(part 1 of 2)
# Autodesk Inventor assembly: Raspberry Pi 3
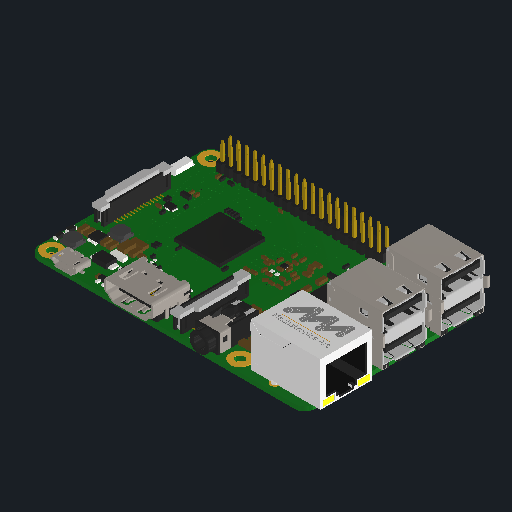
[picture p0: Inventor's stored thumbnail of the model, 512x512]
Saved by Autodesk Inventor 2023 (Build 270158000, 158)
## iProperties
Created: 2016-12-17
Part Number: Raspberry Pi 3
Description: STEP AP214
Document SubType Name: Assembly
Designer: Manuel
Sending System: SolidWorks 2016
Preprocessor: SwSTEP 2.0
Title: Raspberry Pi 3.STEP
Revision Number: ANY
## Documents named in this file (328)
- C:\workspace\Studium\WST\opcua_netzwerk\Entwicklung Knoten\3D Modell\Raspberry Pi 3B\Raspberry Pi 3.iam
- C:\workspace\Studium\WST\opcua_netzwerk\Entwicklung Knoten\3D Modell\Raspberry Pi 3B\Raspberry Pi 3157.ipt
- C:\workspace\Studium\WST\opcua_netzwerk\Entwicklung Knoten\3D Modell\Raspberry Pi 3B\Raspberry Pi 3242.ipt
- C:\workspace\Studium\WST\opcua_netzwerk\Entwicklung Knoten\3D Modell\Raspberry Pi 3B\Raspberry Pi 3266.ipt
- C:\workspace\Studium\WST\opcua_netzwerk\Entwicklung Knoten\3D Modell\Raspberry Pi 3B\raspberry_pi_3(bar_180_2x20).ipt
- C:\workspace\Studium\WST\opcua_netzwerk\Entwicklung Knoten\3D Modell\Raspberry Pi 3B\RPi3_ModelB v1.iam
- C:\workspace\Studium\WST\opcua_netzwerk\Entwicklung Knoten\3D Modell\Raspberry Pi 3B\Raspberry Pi 312.ipt
- C:\workspace\Studium\WST\opcua_netzwerk\Entwicklung Knoten\3D Modell\Raspberry Pi 3B\Raspberry Pi 314.ipt
- C:\workspace\Studium\WST\opcua_netzwerk\Entwicklung Knoten\3D Modell\Raspberry Pi 3B\Raspberry Pi 3172.ipt
- C:\workspace\Studium\WST\opcua_netzwerk\Entwicklung Knoten\3D Modell\Raspberry Pi 3B\Raspberry Pi 3173.ipt
- C:\workspace\Studium\WST\opcua_netzwerk\Entwicklung Knoten\3D Modell\Raspberry Pi 3B\Raspberry Pi 3174.ipt
- C:\workspace\Studium\WST\opcua_netzwerk\Entwicklung Knoten\3D Modell\Raspberry Pi 3B\Raspberry Pi 3175.ipt
- C:\workspace\Studium\WST\opcua_netzwerk\Entwicklung Knoten\3D Modell\Raspberry Pi 3B\Raspberry Pi 3176.ipt
- C:\workspace\Studium\WST\opcua_netzwerk\Entwicklung Knoten\3D Modell\Raspberry Pi 3B\Raspberry Pi 3177.ipt
- C:\workspace\Studium\WST\opcua_netzwerk\Entwicklung Knoten\3D Modell\Raspberry Pi 3B\Raspberry Pi 3178.ipt
- C:\workspace\Studium\WST\opcua_netzwerk\Entwicklung Knoten\3D Modell\Raspberry Pi 3B\Raspberry Pi 3179.ipt
- C:\workspace\Studium\WST\opcua_netzwerk\Entwicklung Knoten\3D Modell\Raspberry Pi 3B\Raspberry Pi 3180.ipt
- C:\workspace\Studium\WST\opcua_netzwerk\Entwicklung Knoten\3D Modell\Raspberry Pi 3B\Raspberry Pi 3181.ipt
- C:\workspace\Studium\WST\opcua_netzwerk\Entwicklung Knoten\3D Modell\Raspberry Pi 3B\Raspberry Pi 3182.ipt
- C:\workspace\Studium\WST\opcua_netzwerk\Entwicklung Knoten\3D Modell\Raspberry Pi 3B\Raspberry Pi 3183.ipt
- C:\workspace\Studium\WST\opcua_netzwerk\Entwicklung Knoten\3D Modell\Raspberry Pi 3B\Raspberry Pi 3184.ipt
- C:\workspace\Studium\WST\opcua_netzwerk\Entwicklung Knoten\3D Modell\Raspberry Pi 3B\Raspberry Pi 3185.ipt
- C:\workspace\Studium\WST\opcua_netzwerk\Entwicklung Knoten\3D Modell\Raspberry Pi 3B\Raspberry Pi 3186.ipt
- C:\workspace\Studium\WST\opcua_netzwerk\Entwicklung Knoten\3D Modell\Raspberry Pi 3B\Raspberry Pi 3187.ipt
- C:\workspace\Studium\WST\opcua_netzwerk\Entwicklung Knoten\3D Modell\Raspberry Pi 3B\Raspberry Pi 3188.ipt
- C:\workspace\Studium\WST\opcua_netzwerk\Entwicklung Knoten\3D Modell\Raspberry Pi 3B\Raspberry Pi 3189.ipt
- C:\workspace\Studium\WST\opcua_netzwerk\Entwicklung Knoten\3D Modell\Raspberry Pi 3B\Raspberry Pi 3190.ipt
- C:\workspace\Studium\WST\opcua_netzwerk\Entwicklung Knoten\3D Modell\Raspberry Pi 3B\Raspberry Pi 3191.ipt
- C:\workspace\Studium\WST\opcua_netzwerk\Entwicklung Knoten\3D Modell\Raspberry Pi 3B\Raspberry Pi 3192.ipt
- C:\workspace\Studium\WST\opcua_netzwerk\Entwicklung Knoten\3D Modell\Raspberry Pi 3B\Raspberry Pi 3193.ipt
- C:\workspace\Studium\WST\opcua_netzwerk\Entwicklung Knoten\3D Modell\Raspberry Pi 3B\Raspberry Pi 3194.ipt
- C:\workspace\Studium\WST\opcua_netzwerk\Entwicklung Knoten\3D Modell\Raspberry Pi 3B\Raspberry Pi 3195.ipt
- C:\workspace\Studium\WST\opcua_netzwerk\Entwicklung Knoten\3D Modell\Raspberry Pi 3B\Raspberry Pi 3196.ipt
- C:\workspace\Studium\WST\opcua_netzwerk\Entwicklung Knoten\3D Modell\Raspberry Pi 3B\Raspberry Pi 3197.ipt
- C:\workspace\Studium\WST\opcua_netzwerk\Entwicklung Knoten\3D Modell\Raspberry Pi 3B\Raspberry Pi 3198.ipt
- C:\workspace\Studium\WST\opcua_netzwerk\Entwicklung Knoten\3D Modell\Raspberry Pi 3B\Raspberry Pi 3199.ipt
- C:\workspace\Studium\WST\opcua_netzwerk\Entwicklung Knoten\3D Modell\Raspberry Pi 3B\Raspberry Pi 3200.ipt
- C:\workspace\Studium\WST\opcua_netzwerk\Entwicklung Knoten\3D Modell\Raspberry Pi 3B\Raspberry Pi 3201.ipt
- C:\workspace\Studium\WST\opcua_netzwerk\Entwicklung Knoten\3D Modell\Raspberry Pi 3B\Raspberry Pi 3202.ipt
- C:\workspace\Studium\WST\opcua_netzwerk\Entwicklung Knoten\3D Modell\Raspberry Pi 3B\Raspberry Pi 3203.ipt
- C:\workspace\Studium\WST\opcua_netzwerk\Entwicklung Knoten\3D Modell\Raspberry Pi 3B\Raspberry Pi 3204.ipt
- C:\workspace\Studium\WST\opcua_netzwerk\Entwicklung Knoten\3D Modell\Raspberry Pi 3B\Raspberry Pi 3205.ipt
- C:\workspace\Studium\WST\opcua_netzwerk\Entwicklung Knoten\3D Modell\Raspberry Pi 3B\Raspberry Pi 3206.ipt
- C:\workspace\Studium\WST\opcua_netzwerk\Entwicklung Knoten\3D Modell\Raspberry Pi 3B\Raspberry Pi 3207.ipt
- C:\workspace\Studium\WST\opcua_netzwerk\Entwicklung Knoten\3D Modell\Raspberry Pi 3B\Raspberry Pi 3208.ipt
- C:\workspace\Studium\WST\opcua_netzwerk\Entwicklung Knoten\3D Modell\Raspberry Pi 3B\Raspberry Pi 3209.ipt
- C:\workspace\Studium\WST\opcua_netzwerk\Entwicklung Knoten\3D Modell\Raspberry Pi 3B\Raspberry Pi 3210.ipt
- C:\workspace\Studium\WST\opcua_netzwerk\Entwicklung Knoten\3D Modell\Raspberry Pi 3B\Raspberry Pi 3211.ipt
- C:\workspace\Studium\WST\opcua_netzwerk\Entwicklung Knoten\3D Modell\Raspberry Pi 3B\Raspberry Pi 3212.ipt
- C:\workspace\Studium\WST\opcua_netzwerk\Entwicklung Knoten\3D Modell\Raspberry Pi 3B\Raspberry Pi 3213.ipt
- C:\workspace\Studium\WST\opcua_netzwerk\Entwicklung Knoten\3D Modell\Raspberry Pi 3B\Raspberry Pi 3214.ipt
- C:\workspace\Studium\WST\opcua_netzwerk\Entwicklung Knoten\3D Modell\Raspberry Pi 3B\Raspberry Pi 3215.ipt
- C:\workspace\Studium\WST\opcua_netzwerk\Entwicklung Knoten\3D Modell\Raspberry Pi 3B\Raspberry Pi 3216.ipt
- C:\workspace\Studium\WST\opcua_netzwerk\Entwicklung Knoten\3D Modell\Raspberry Pi 3B\Raspberry Pi 3217.ipt
- C:\workspace\Studium\WST\opcua_netzwerk\Entwicklung Knoten\3D Modell\Raspberry Pi 3B\Raspberry Pi 3218.ipt
- C:\workspace\Studium\WST\opcua_netzwerk\Entwicklung Knoten\3D Modell\Raspberry Pi 3B\Raspberry Pi 3219.ipt
- C:\workspace\Studium\WST\opcua_netzwerk\Entwicklung Knoten\3D Modell\Raspberry Pi 3B\Raspberry Pi 3220.ipt
- C:\workspace\Studium\WST\opcua_netzwerk\Entwicklung Knoten\3D Modell\Raspberry Pi 3B\Raspberry Pi 3221.ipt
- C:\workspace\Studium\WST\opcua_netzwerk\Entwicklung Knoten\3D Modell\Raspberry Pi 3B\Raspberry Pi 3222.ipt
- C:\workspace\Studium\WST\opcua_netzwerk\Entwicklung Knoten\3D Modell\Raspberry Pi 3B\Raspberry Pi 3223.ipt
- C:\workspace\Studium\WST\opcua_netzwerk\Entwicklung Knoten\3D Modell\Raspberry Pi 3B\Raspberry Pi 3224.ipt
- C:\workspace\Studium\WST\opcua_netzwerk\Entwicklung Knoten\3D Modell\Raspberry Pi 3B\Raspberry Pi 3225.ipt
- C:\workspace\Studium\WST\opcua_netzwerk\Entwicklung Knoten\3D Modell\Raspberry Pi 3B\Raspberry Pi 3226.ipt
- C:\workspace\Studium\WST\opcua_netzwerk\Entwicklung Knoten\3D Modell\Raspberry Pi 3B\Raspberry Pi 3227.ipt
- C:\workspace\Studium\WST\opcua_netzwerk\Entwicklung Knoten\3D Modell\Raspberry Pi 3B\Raspberry Pi 3228.ipt
- C:\workspace\Studium\WST\opcua_netzwerk\Entwicklung Knoten\3D Modell\Raspberry Pi 3B\Raspberry Pi 3229.ipt
- C:\workspace\Studium\WST\opcua_netzwerk\Entwicklung Knoten\3D Modell\Raspberry Pi 3B\Raspberry Pi 3230.ipt
- C:\workspace\Studium\WST\opcua_netzwerk\Entwicklung Knoten\3D Modell\Raspberry Pi 3B\Raspberry Pi 3231.ipt
- C:\workspace\Studium\WST\opcua_netzwerk\Entwicklung Knoten\3D Modell\Raspberry Pi 3B\Raspberry Pi 3232.ipt
- C:\workspace\Studium\WST\opcua_netzwerk\Entwicklung Knoten\3D Modell\Raspberry Pi 3B\Raspberry Pi 3233.ipt
- C:\workspace\Studium\WST\opcua_netzwerk\Entwicklung Knoten\3D Modell\Raspberry Pi 3B\Raspberry Pi 3234.ipt
- C:\workspace\Studium\WST\opcua_netzwerk\Entwicklung Knoten\3D Modell\Raspberry Pi 3B\Raspberry Pi 3235.ipt
- C:\workspace\Studium\WST\opcua_netzwerk\Entwicklung Knoten\3D Modell\Raspberry Pi 3B\Raspberry Pi 31.ipt
- C:\workspace\Studium\WST\opcua_netzwerk\Entwicklung Knoten\3D Modell\Raspberry Pi 3B\Raspberry Pi 32.ipt
- C:\workspace\Studium\WST\opcua_netzwerk\Entwicklung Knoten\3D Modell\Raspberry Pi 3B\Raspberry Pi 33.ipt
- C:\workspace\Studium\WST\opcua_netzwerk\Entwicklung Knoten\3D Modell\Raspberry Pi 3B\Raspberry Pi 34.ipt
- C:\workspace\Studium\WST\opcua_netzwerk\Entwicklung Knoten\3D Modell\Raspberry Pi 3B\Raspberry Pi 35.ipt
- C:\workspace\Studium\WST\opcua_netzwerk\Entwicklung Knoten\3D Modell\Raspberry Pi 3B\Raspberry Pi 36.ipt
- C:\workspace\Studium\WST\opcua_netzwerk\Entwicklung Knoten\3D Modell\Raspberry Pi 3B\Raspberry Pi 37.ipt
- C:\workspace\Studium\WST\opcua_netzwerk\Entwicklung Knoten\3D Modell\Raspberry Pi 3B\Raspberry Pi 38.ipt
- C:\workspace\Studium\WST\opcua_netzwerk\Entwicklung Knoten\3D Modell\Raspberry Pi 3B\Raspberry Pi 39.ipt
- C:\workspace\Studium\WST\opcua_netzwerk\Entwicklung Knoten\3D Modell\Raspberry Pi 3B\Raspberry Pi 310.ipt
- C:\workspace\Studium\WST\opcua_netzwerk\Entwicklung Knoten\3D Modell\Raspberry Pi 3B\Raspberry Pi 311.ipt
- C:\workspace\Studium\WST\opcua_netzwerk\Entwicklung Knoten\3D Modell\Raspberry Pi 3B\Raspberry Pi 313.ipt
- C:\workspace\Studium\WST\opcua_netzwerk\Entwicklung Knoten\3D Modell\Raspberry Pi 3B\Raspberry Pi 315.ipt
- C:\workspace\Studium\WST\opcua_netzwerk\Entwicklung Knoten\3D Modell\Raspberry Pi 3B\Raspberry Pi 316.ipt
- C:\workspace\Studium\WST\opcua_netzwerk\Entwicklung Knoten\3D Modell\Raspberry Pi 3B\Raspberry Pi 317.ipt
- C:\workspace\Studium\WST\opcua_netzwerk\Entwicklung Knoten\3D Modell\Raspberry Pi 3B\Raspberry Pi 318.ipt
- C:\workspace\Studium\WST\opcua_netzwerk\Entwicklung Knoten\3D Modell\Raspberry Pi 3B\Raspberry Pi 319.ipt
- C:\workspace\Studium\WST\opcua_netzwerk\Entwicklung Knoten\3D Modell\Raspberry Pi 3B\Raspberry Pi 320.ipt
- C:\workspace\Studium\WST\opcua_netzwerk\Entwicklung Knoten\3D Modell\Raspberry Pi 3B\Raspberry Pi 322.ipt
- C:\workspace\Studium\WST\opcua_netzwerk\Entwicklung Knoten\3D Modell\Raspberry Pi 3B\Raspberry Pi 323.ipt
- C:\workspace\Studium\WST\opcua_netzwerk\Entwicklung Knoten\3D Modell\Raspberry Pi 3B\Raspberry Pi 324.ipt
- C:\workspace\Studium\WST\opcua_netzwerk\Entwicklung Knoten\3D Modell\Raspberry Pi 3B\Raspberry Pi 325.ipt
- C:\workspace\Studium\WST\opcua_netzwerk\Entwicklung Knoten\3D Modell\Raspberry Pi 3B\Raspberry Pi 326.ipt
- C:\workspace\Studium\WST\opcua_netzwerk\Entwicklung Knoten\3D Modell\Raspberry Pi 3B\Raspberry Pi 327.ipt
- C:\workspace\Studium\WST\opcua_netzwerk\Entwicklung Knoten\3D Modell\Raspberry Pi 3B\Raspberry Pi 328.ipt
- C:\workspace\Studium\WST\opcua_netzwerk\Entwicklung Knoten\3D Modell\Raspberry Pi 3B\Raspberry Pi 329.ipt
- C:\workspace\Studium\WST\opcua_netzwerk\Entwicklung Knoten\3D Modell\Raspberry Pi 3B\Raspberry Pi 330.ipt
- C:\workspace\Studium\WST\opcua_netzwerk\Entwicklung Knoten\3D Modell\Raspberry Pi 3B\Raspberry Pi 331.ipt
- C:\workspace\Studium\WST\opcua_netzwerk\Entwicklung Knoten\3D Modell\Raspberry Pi 3B\Raspberry Pi 332.ipt
- C:\workspace\Studium\WST\opcua_netzwerk\Entwicklung Knoten\3D Modell\Raspberry Pi 3B\Raspberry Pi 333.ipt
- C:\workspace\Studium\WST\opcua_netzwerk\Entwicklung Knoten\3D Modell\Raspberry Pi 3B\Raspberry Pi 334.ipt
- C:\workspace\Studium\WST\opcua_netzwerk\Entwicklung Knoten\3D Modell\Raspberry Pi 3B\Raspberry Pi 335.ipt
- C:\workspace\Studium\WST\opcua_netzwerk\Entwicklung Knoten\3D Modell\Raspberry Pi 3B\Raspberry Pi 336.ipt
- C:\workspace\Studium\WST\opcua_netzwerk\Entwicklung Knoten\3D Modell\Raspberry Pi 3B\Raspberry Pi 337.ipt
- C:\workspace\Studium\WST\opcua_netzwerk\Entwicklung Knoten\3D Modell\Raspberry Pi 3B\Raspberry Pi 338.ipt
- C:\workspace\Studium\WST\opcua_netzwerk\Entwicklung Knoten\3D Modell\Raspberry Pi 3B\Raspberry Pi 339.ipt
- C:\workspace\Studium\WST\opcua_netzwerk\Entwicklung Knoten\3D Modell\Raspberry Pi 3B\Raspberry Pi 340.ipt
- C:\workspace\Studium\WST\opcua_netzwerk\Entwicklung Knoten\3D Modell\Raspberry Pi 3B\Raspberry Pi 341.ipt
- C:\workspace\Studium\WST\opcua_netzwerk\Entwicklung Knoten\3D Modell\Raspberry Pi 3B\Raspberry Pi 342.ipt
- C:\workspace\Studium\WST\opcua_netzwerk\Entwicklung Knoten\3D Modell\Raspberry Pi 3B\Raspberry Pi 343.ipt
- C:\workspace\Studium\WST\opcua_netzwerk\Entwicklung Knoten\3D Modell\Raspberry Pi 3B\Raspberry Pi 344.ipt
- C:\workspace\Studium\WST\opcua_netzwerk\Entwicklung Knoten\3D Modell\Raspberry Pi 3B\Raspberry Pi 345.ipt
- C:\workspace\Studium\WST\opcua_netzwerk\Entwicklung Knoten\3D Modell\Raspberry Pi 3B\Raspberry Pi 346.ipt
- C:\workspace\Studium\WST\opcua_netzwerk\Entwicklung Knoten\3D Modell\Raspberry Pi 3B\Raspberry Pi 347.ipt
- C:\workspace\Studium\WST\opcua_netzwerk\Entwicklung Knoten\3D Modell\Raspberry Pi 3B\Raspberry Pi 348.ipt
- C:\workspace\Studium\WST\opcua_netzwerk\Entwicklung Knoten\3D Modell\Raspberry Pi 3B\Raspberry Pi 349.ipt
- C:\workspace\Studium\WST\opcua_netzwerk\Entwicklung Knoten\3D Modell\Raspberry Pi 3B\Raspberry Pi 350.ipt
- C:\workspace\Studium\WST\opcua_netzwerk\Entwicklung Knoten\3D Modell\Raspberry Pi 3B\Raspberry Pi 351.ipt
- C:\workspace\Studium\WST\opcua_netzwerk\Entwicklung Knoten\3D Modell\Raspberry Pi 3B\Raspberry Pi 352.ipt
- C:\workspace\Studium\WST\opcua_netzwerk\Entwicklung Knoten\3D Modell\Raspberry Pi 3B\Raspberry Pi 353.ipt
- C:\workspace\Studium\WST\opcua_netzwerk\Entwicklung Knoten\3D Modell\Raspberry Pi 3B\Raspberry Pi 354.ipt
- C:\workspace\Studium\WST\opcua_netzwerk\Entwicklung Knoten\3D Modell\Raspberry Pi 3B\Raspberry Pi 355.ipt
- C:\workspace\Studium\WST\opcua_netzwerk\Entwicklung Knoten\3D Modell\Raspberry Pi 3B\Raspberry Pi 356.ipt
- C:\workspace\Studium\WST\opcua_netzwerk\Entwicklung Knoten\3D Modell\Raspberry Pi 3B\Raspberry Pi 357.ipt
- C:\workspace\Studium\WST\opcua_netzwerk\Entwicklung Knoten\3D Modell\Raspberry Pi 3B\Raspberry Pi 358.ipt
- C:\workspace\Studium\WST\opcua_netzwerk\Entwicklung Knoten\3D Modell\Raspberry Pi 3B\Raspberry Pi 359.ipt
- C:\workspace\Studium\WST\opcua_netzwerk\Entwicklung Knoten\3D Modell\Raspberry Pi 3B\Raspberry Pi 360.ipt
- C:\workspace\Studium\WST\opcua_netzwerk\Entwicklung Knoten\3D Modell\Raspberry Pi 3B\Raspberry Pi 361.ipt
- C:\workspace\Studium\WST\opcua_netzwerk\Entwicklung Knoten\3D Modell\Raspberry Pi 3B\Raspberry Pi 362.ipt
- C:\workspace\Studium\WST\opcua_netzwerk\Entwicklung Knoten\3D Modell\Raspberry Pi 3B\Raspberry Pi 363.ipt
- C:\workspace\Studium\WST\opcua_netzwerk\Entwicklung Knoten\3D Modell\Raspberry Pi 3B\Raspberry Pi 364.ipt
- C:\workspace\Studium\WST\opcua_netzwerk\Entwicklung Knoten\3D Modell\Raspberry Pi 3B\Raspberry Pi 365.ipt
- C:\workspace\Studium\WST\opcua_netzwerk\Entwicklung Knoten\3D Modell\Raspberry Pi 3B\Raspberry Pi 366.ipt
- C:\workspace\Studium\WST\opcua_netzwerk\Entwicklung Knoten\3D Modell\Raspberry Pi 3B\Raspberry Pi 367.ipt
- C:\workspace\Studium\WST\opcua_netzwerk\Entwicklung Knoten\3D Modell\Raspberry Pi 3B\Raspberry Pi 368.ipt
- C:\workspace\Studium\WST\opcua_netzwerk\Entwicklung Knoten\3D Modell\Raspberry Pi 3B\Raspberry Pi 369.ipt
- C:\workspace\Studium\WST\opcua_netzwerk\Entwicklung Knoten\3D Modell\Raspberry Pi 3B\Raspberry Pi 370.ipt
- C:\workspace\Studium\WST\opcua_netzwerk\Entwicklung Knoten\3D Modell\Raspberry Pi 3B\Raspberry Pi 371.ipt
- C:\workspace\Studium\WST\opcua_netzwerk\Entwicklung Knoten\3D Modell\Raspberry Pi 3B\Raspberry Pi 372.ipt
- C:\workspace\Studium\WST\opcua_netzwerk\Entwicklung Knoten\3D Modell\Raspberry Pi 3B\Raspberry Pi 373.ipt
- C:\workspace\Studium\WST\opcua_netzwerk\Entwicklung Knoten\3D Modell\Raspberry Pi 3B\Raspberry Pi 374.ipt
- C:\workspace\Studium\WST\opcua_netzwerk\Entwicklung Knoten\3D Modell\Raspberry Pi 3B\Raspberry Pi 375.ipt
- C:\workspace\Studium\WST\opcua_netzwerk\Entwicklung Knoten\3D Modell\Raspberry Pi 3B\Raspberry Pi 376.ipt
- C:\workspace\Studium\WST\opcua_netzwerk\Entwicklung Knoten\3D Modell\Raspberry Pi 3B\Raspberry Pi 377.ipt
- C:\workspace\Studium\WST\opcua_netzwerk\Entwicklung Knoten\3D Modell\Raspberry Pi 3B\Raspberry Pi 378.ipt
- C:\workspace\Studium\WST\opcua_netzwerk\Entwicklung Knoten\3D Modell\Raspberry Pi 3B\Raspberry Pi 379.ipt
- C:\workspace\Studium\WST\opcua_netzwerk\Entwicklung Knoten\3D Modell\Raspberry Pi 3B\Raspberry Pi 380.ipt
- C:\workspace\Studium\WST\opcua_netzwerk\Entwicklung Knoten\3D Modell\Raspberry Pi 3B\Raspberry Pi 381.ipt
- C:\workspace\Studium\WST\opcua_netzwerk\Entwicklung Knoten\3D Modell\Raspberry Pi 3B\Raspberry Pi 382.ipt
- C:\workspace\Studium\WST\opcua_netzwerk\Entwicklung Knoten\3D Modell\Raspberry Pi 3B\Raspberry Pi 383.ipt
- C:\workspace\Studium\WST\opcua_netzwerk\Entwicklung Knoten\3D Modell\Raspberry Pi 3B\Raspberry Pi 385.ipt
- C:\workspace\Studium\WST\opcua_netzwerk\Entwicklung Knoten\3D Modell\Raspberry Pi 3B\Raspberry Pi 386.ipt
- C:\workspace\Studium\WST\opcua_netzwerk\Entwicklung Knoten\3D Modell\Raspberry Pi 3B\Raspberry Pi 387.ipt
- C:\workspace\Studium\WST\opcua_netzwerk\Entwicklung Knoten\3D Modell\Raspberry Pi 3B\Raspberry Pi 388.ipt
- C:\workspace\Studium\WST\opcua_netzwerk\Entwicklung Knoten\3D Modell\Raspberry Pi 3B\Raspberry Pi 390.ipt
- C:\workspace\Studium\WST\opcua_netzwerk\Entwicklung Knoten\3D Modell\Raspberry Pi 3B\Raspberry Pi 391.ipt
- C:\workspace\Studium\WST\opcua_netzwerk\Entwicklung Knoten\3D Modell\Raspberry Pi 3B\Raspberry Pi 393.ipt
- C:\workspace\Studium\WST\opcua_netzwerk\Entwicklung Knoten\3D Modell\Raspberry Pi 3B\Raspberry Pi 394.ipt
- C:\workspace\Studium\WST\opcua_netzwerk\Entwicklung Knoten\3D Modell\Raspberry Pi 3B\Raspberry Pi 395.ipt
- C:\workspace\Studium\WST\opcua_netzwerk\Entwicklung Knoten\3D Modell\Raspberry Pi 3B\Raspberry Pi 396.ipt
- C:\workspace\Studium\WST\opcua_netzwerk\Entwicklung Knoten\3D Modell\Raspberry Pi 3B\Raspberry Pi 397.ipt
- C:\workspace\Studium\WST\opcua_netzwerk\Entwicklung Knoten\3D Modell\Raspberry Pi 3B\Raspberry Pi 398.ipt
- C:\workspace\Studium\WST\opcua_netzwerk\Entwicklung Knoten\3D Modell\Raspberry Pi 3B\Raspberry Pi 399.ipt
- C:\workspace\Studium\WST\opcua_netzwerk\Entwicklung Knoten\3D Modell\Raspberry Pi 3B\Raspberry Pi 3100.ipt
- C:\workspace\Studium\WST\opcua_netzwerk\Entwicklung Knoten\3D Modell\Raspberry Pi 3B\Raspberry Pi 3101.ipt
- C:\workspace\Studium\WST\opcua_netzwerk\Entwicklung Knoten\3D Modell\Raspberry Pi 3B\Raspberry Pi 3102.ipt
- C:\workspace\Studium\WST\opcua_netzwerk\Entwicklung Knoten\3D Modell\Raspberry Pi 3B\Raspberry Pi 3103.ipt
- C:\workspace\Studium\WST\opcua_netzwerk\Entwicklung Knoten\3D Modell\Raspberry Pi 3B\Raspberry Pi 3104.ipt
- C:\workspace\Studium\WST\opcua_netzwerk\Entwicklung Knoten\3D Modell\Raspberry Pi 3B\Raspberry Pi 3105.ipt
- C:\workspace\Studium\WST\opcua_netzwerk\Entwicklung Knoten\3D Modell\Raspberry Pi 3B\Raspberry Pi 3106.ipt
- C:\workspace\Studium\WST\opcua_netzwerk\Entwicklung Knoten\3D Modell\Raspberry Pi 3B\Raspberry Pi 3107.ipt
- C:\workspace\Studium\WST\opcua_netzwerk\Entwicklung Knoten\3D Modell\Raspberry Pi 3B\Raspberry Pi 3108.ipt
- C:\workspace\Studium\WST\opcua_netzwerk\Entwicklung Knoten\3D Modell\Raspberry Pi 3B\Raspberry Pi 3109.ipt
- C:\workspace\Studium\WST\opcua_netzwerk\Entwicklung Knoten\3D Modell\Raspberry Pi 3B\Raspberry Pi 3110.ipt
- C:\workspace\Studium\WST\opcua_netzwerk\Entwicklung Knoten\3D Modell\Raspberry Pi 3B\Raspberry Pi 3111.ipt
- C:\workspace\Studium\WST\opcua_netzwerk\Entwicklung Knoten\3D Modell\Raspberry Pi 3B\Raspberry Pi 3112.ipt
- C:\workspace\Studium\WST\opcua_netzwerk\Entwicklung Knoten\3D Modell\Raspberry Pi 3B\Raspberry Pi 3113.ipt
- C:\workspace\Studium\WST\opcua_netzwerk\Entwicklung Knoten\3D Modell\Raspberry Pi 3B\Raspberry Pi 3114.ipt
- C:\workspace\Studium\WST\opcua_netzwerk\Entwicklung Knoten\3D Modell\Raspberry Pi 3B\Raspberry Pi 3115.ipt
- C:\workspace\Studium\WST\opcua_netzwerk\Entwicklung Knoten\3D Modell\Raspberry Pi 3B\Raspberry Pi 3116.ipt
- C:\workspace\Studium\WST\opcua_netzwerk\Entwicklung Knoten\3D Modell\Raspberry Pi 3B\Raspberry Pi 3117.ipt
- C:\workspace\Studium\WST\opcua_netzwerk\Entwicklung Knoten\3D Modell\Raspberry Pi 3B\Raspberry Pi 3118.ipt
- C:\workspace\Studium\WST\opcua_netzwerk\Entwicklung Knoten\3D Modell\Raspberry Pi 3B\Raspberry Pi 3119.ipt
- C:\workspace\Studium\WST\opcua_netzwerk\Entwicklung Knoten\3D Modell\Raspberry Pi 3B\Raspberry Pi 3120.ipt
- C:\workspace\Studium\WST\opcua_netzwerk\Entwicklung Knoten\3D Modell\Raspberry Pi 3B\Raspberry Pi 3121.ipt
- C:\workspace\Studium\WST\opcua_netzwerk\Entwicklung Knoten\3D Modell\Raspberry Pi 3B\Raspberry Pi 3122.ipt
- C:\workspace\Studium\WST\opcua_netzwerk\Entwicklung Knoten\3D Modell\Raspberry Pi 3B\Raspberry Pi 3123.ipt
- C:\workspace\Studium\WST\opcua_netzwerk\Entwicklung Knoten\3D Modell\Raspberry Pi 3B\Raspberry Pi 3124.ipt
- C:\workspace\Studium\WST\opcua_netzwerk\Entwicklung Knoten\3D Modell\Raspberry Pi 3B\Raspberry Pi 3125.ipt
- C:\workspace\Studium\WST\opcua_netzwerk\Entwicklung Knoten\3D Modell\Raspberry Pi 3B\Raspberry Pi 3126.ipt
- C:\workspace\Studium\WST\opcua_netzwerk\Entwicklung Knoten\3D Modell\Raspberry Pi 3B\Raspberry Pi 3127.ipt
- C:\workspace\Studium\WST\opcua_netzwerk\Entwicklung Knoten\3D Modell\Raspberry Pi 3B\Raspberry Pi 3128.ipt
- C:\workspace\Studium\WST\opcua_netzwerk\Entwicklung Knoten\3D Modell\Raspberry Pi 3B\Raspberry Pi 3129.ipt
- C:\workspace\Studium\WST\opcua_netzwerk\Entwicklung Knoten\3D Modell\Raspberry Pi 3B\Raspberry Pi 3130.ipt
- C:\workspace\Studium\WST\opcua_netzwerk\Entwicklung Knoten\3D Modell\Raspberry Pi 3B\Raspberry Pi 3131.ipt
- C:\workspace\Studium\WST\opcua_netzwerk\Entwicklung Knoten\3D Modell\Raspberry Pi 3B\Raspberry Pi 3132.ipt
- C:\workspace\Studium\WST\opcua_netzwerk\Entwicklung Knoten\3D Modell\Raspberry Pi 3B\Raspberry Pi 3133.ipt
- C:\workspace\Studium\WST\opcua_netzwerk\Entwicklung Knoten\3D Modell\Raspberry Pi 3B\Raspberry Pi 3134.ipt
- C:\workspace\Studium\WST\opcua_netzwerk\Entwicklung Knoten\3D Modell\Raspberry Pi 3B\Raspberry Pi 3135.ipt
- C:\workspace\Studium\WST\opcua_netzwerk\Entwicklung Knoten\3D Modell\Raspberry Pi 3B\Raspberry Pi 3137.ipt
- C:\workspace\Studium\WST\opcua_netzwerk\Entwicklung Knoten\3D Modell\Raspberry Pi 3B\Raspberry Pi 3138.ipt
- C:\workspace\Studium\WST\opcua_netzwerk\Entwicklung Knoten\3D Modell\Raspberry Pi 3B\Raspberry Pi 3139.ipt
- C:\workspace\Studium\WST\opcua_netzwerk\Entwicklung Knoten\3D Modell\Raspberry Pi 3B\Raspberry Pi 3140.ipt
- C:\workspace\Studium\WST\opcua_netzwerk\Entwicklung Knoten\3D Modell\Raspberry Pi 3B\Raspberry Pi 3141.ipt
- C:\workspace\Studium\WST\opcua_netzwerk\Entwicklung Knoten\3D Modell\Raspberry Pi 3B\Raspberry Pi 3142.ipt
- C:\workspace\Studium\WST\opcua_netzwerk\Entwicklung Knoten\3D Modell\Raspberry Pi 3B\Raspberry Pi 3143.ipt
- C:\workspace\Studium\WST\opcua_netzwerk\Entwicklung Knoten\3D Modell\Raspberry Pi 3B\Raspberry Pi 3144.ipt
- C:\workspace\Studium\WST\opcua_netzwerk\Entwicklung Knoten\3D Modell\Raspberry Pi 3B\Raspberry Pi 3146.ipt
- C:\workspace\Studium\WST\opcua_netzwerk\Entwicklung Knoten\3D Modell\Raspberry Pi 3B\Raspberry Pi 3147.ipt
- C:\workspace\Studium\WST\opcua_netzwerk\Entwicklung Knoten\3D Modell\Raspberry Pi 3B\Raspberry Pi 3149.ipt
- C:\workspace\Studium\WST\opcua_netzwerk\Entwicklung Knoten\3D Modell\Raspberry Pi 3B\Raspberry Pi 3150.ipt
- C:\workspace\Studium\WST\opcua_netzwerk\Entwicklung Knoten\3D Modell\Raspberry Pi 3B\Raspberry Pi 3151.ipt
- C:\workspace\Studium\WST\opcua_netzwerk\Entwicklung Knoten\3D Modell\Raspberry Pi 3B\Raspberry Pi 3152.ipt
- C:\workspace\Studium\WST\opcua_netzwerk\Entwicklung Knoten\3D Modell\Raspberry Pi 3B\Raspberry Pi 3153.ipt
- C:\workspace\Studium\WST\opcua_netzwerk\Entwicklung Knoten\3D Modell\Raspberry Pi 3B\Raspberry Pi 3154.ipt
- C:\workspace\Studium\WST\opcua_netzwerk\Entwicklung Knoten\3D Modell\Raspberry Pi 3B\Raspberry Pi 3155.ipt
- C:\workspace\Studium\WST\opcua_netzwerk\Entwicklung Knoten\3D Modell\Raspberry Pi 3B\Raspberry Pi 3156.ipt
- C:\workspace\Studium\WST\opcua_netzwerk\Entwicklung Knoten\3D Modell\Raspberry Pi 3B\Raspberry Pi 3158.ipt
- C:\workspace\Studium\WST\opcua_netzwerk\Entwicklung Knoten\3D Modell\Raspberry Pi 3B\Raspberry Pi 3159.ipt
- C:\workspace\Studium\WST\opcua_netzwerk\Entwicklung Knoten\3D Modell\Raspberry Pi 3B\Raspberry Pi 3160.ipt
- C:\workspace\Studium\WST\opcua_netzwerk\Entwicklung Knoten\3D Modell\Raspberry Pi 3B\Raspberry Pi 3161.ipt
- C:\workspace\Studium\WST\opcua_netzwerk\Entwicklung Knoten\3D Modell\Raspberry Pi 3B\Raspberry Pi 3162.ipt
- C:\workspace\Studium\WST\opcua_netzwerk\Entwicklung Knoten\3D Modell\Raspberry Pi 3B\Raspberry Pi 3163.ipt
- C:\workspace\Studium\WST\opcua_netzwerk\Entwicklung Knoten\3D Modell\Raspberry Pi 3B\Raspberry Pi 3164.ipt
- C:\workspace\Studium\WST\opcua_netzwerk\Entwicklung Knoten\3D Modell\Raspberry Pi 3B\Raspberry Pi 3165.ipt
- C:\workspace\Studium\WST\opcua_netzwerk\Entwicklung Knoten\3D Modell\Raspberry Pi 3B\Raspberry Pi 3166.ipt
- C:\workspace\Studium\WST\opcua_netzwerk\Entwicklung Knoten\3D Modell\Raspberry Pi 3B\Raspberry Pi 3167.ipt
- C:\workspace\Studium\WST\opcua_netzwerk\Entwicklung Knoten\3D Modell\Raspberry Pi 3B\Raspberry Pi 3168.ipt
- C:\workspace\Studium\WST\opcua_netzwerk\Entwicklung Knoten\3D Modell\Raspberry Pi 3B\Raspberry Pi 3169.ipt
- C:\workspace\Studium\WST\opcua_netzwerk\Entwicklung Knoten\3D Modell\Raspberry Pi 3B\Raspberry Pi 3170.ipt
- C:\workspace\Studium\WST\opcua_netzwerk\Entwicklung Knoten\3D Modell\Raspberry Pi 3B\Raspberry Pi 3171.ipt
- C:\workspace\Studium\WST\opcua_netzwerk\Entwicklung Knoten\3D Modell\Raspberry Pi 3B\Raspberry Pi 3276.ipt
- C:\workspace\Studium\WST\opcua_netzwerk\Entwicklung Knoten\3D Modell\Raspberry Pi 3B\Raspberry Pi 3277.ipt
- C:\workspace\Studium\WST\opcua_netzwerk\Entwicklung Knoten\3D Modell\Raspberry Pi 3B\Raspberry Pi 3278.ipt
- C:\workspace\Studium\WST\opcua_netzwerk\Entwicklung Knoten\3D Modell\Raspberry Pi 3B\Raspberry Pi 3279.ipt
- C:\workspace\Studium\WST\opcua_netzwerk\Entwicklung Knoten\3D Modell\Raspberry Pi 3B\Raspberry Pi 3280.ipt
- C:\workspace\Studium\WST\opcua_netzwerk\Entwicklung Knoten\3D Modell\Raspberry Pi 3B\Raspberry Pi 3281.ipt
- C:\workspace\Studium\WST\opcua_netzwerk\Entwicklung Knoten\3D Modell\Raspberry Pi 3B\Raspberry Pi 3282.ipt
- C:\workspace\Studium\WST\opcua_netzwerk\Entwicklung Knoten\3D Modell\Raspberry Pi 3B\Raspberry Pi 3283.ipt
- C:\workspace\Studium\WST\opcua_netzwerk\Entwicklung Knoten\3D Modell\Raspberry Pi 3B\Raspberry Pi 3284.ipt
- C:\workspace\Studium\WST\opcua_netzwerk\Entwicklung Knoten\3D Modell\Raspberry Pi 3B\Raspberry Pi 3285.ipt
- C:\workspace\Studium\WST\opcua_netzwerk\Entwicklung Knoten\3D Modell\Raspberry Pi 3B\Raspberry Pi 3286.ipt
- C:\workspace\Studium\WST\opcua_netzwerk\Entwicklung Knoten\3D Modell\Raspberry Pi 3B\Raspberry Pi 3287.ipt
- C:\workspace\Studium\WST\opcua_netzwerk\Entwicklung Knoten\3D Modell\Raspberry Pi 3B\Raspberry Pi 3288.ipt
- C:\workspace\Studium\WST\opcua_netzwerk\Entwicklung Knoten\3D Modell\Raspberry Pi 3B\Raspberry Pi 3289.ipt
- C:\workspace\Studium\WST\opcua_netzwerk\Entwicklung Knoten\3D Modell\Raspberry Pi 3B\Raspberry Pi 3290.ipt
- C:\workspace\Studium\WST\opcua_netzwerk\Entwicklung Knoten\3D Modell\Raspberry Pi 3B\Raspberry Pi 3291.ipt
- C:\workspace\Studium\WST\opcua_netzwerk\Entwicklung Knoten\3D Modell\Raspberry Pi 3B\Raspberry Pi 3292.ipt
- C:\workspace\Studium\WST\opcua_netzwerk\Entwicklung Knoten\3D Modell\Raspberry Pi 3B\Raspberry Pi 3293.ipt
- C:\workspace\Studium\WST\opcua_netzwerk\Entwicklung Knoten\3D Modell\Raspberry Pi 3B\Raspberry Pi 3294.ipt
- C:\workspace\Studium\WST\opcua_netzwerk\Entwicklung Knoten\3D Modell\Raspberry Pi 3B\Raspberry Pi 3295.ipt
- C:\workspace\Studium\WST\opcua_netzwerk\Entwicklung Knoten\3D Modell\Raspberry Pi 3B\Raspberry Pi 3296.ipt
- C:\workspace\Studium\WST\opcua_netzwerk\Entwicklung Knoten\3D Modell\Raspberry Pi 3B\Raspberry Pi 3297.ipt
- C:\workspace\Studium\WST\opcua_netzwerk\Entwicklung Knoten\3D Modell\Raspberry Pi 3B\Raspberry Pi 3298.ipt
- C:\workspace\Studium\WST\opcua_netzwerk\Entwicklung Knoten\3D Modell\Raspberry Pi 3B\Raspberry Pi 3299.ipt
- C:\workspace\Studium\WST\opcua_netzwerk\Entwicklung Knoten\3D Modell\Raspberry Pi 3B\Raspberry Pi 3300.ipt
- C:\workspace\Studium\WST\opcua_netzwerk\Entwicklung Knoten\3D Modell\Raspberry Pi 3B\Raspberry Pi 3301.ipt
- C:\workspace\Studium\WST\opcua_netzwerk\Entwicklung Knoten\3D Modell\Raspberry Pi 3B\Raspberry Pi 3302.ipt
- C:\workspace\Studium\WST\opcua_netzwerk\Entwicklung Knoten\3D Modell\Raspberry Pi 3B\Raspberry Pi 3303.ipt
- C:\workspace\Studium\WST\opcua_netzwerk\Entwicklung Knoten\3D Modell\Raspberry Pi 3B\Raspberry Pi 3304.ipt
- C:\workspace\Studium\WST\opcua_netzwerk\Entwicklung Knoten\3D Modell\Raspberry Pi 3B\Raspberry Pi 3305.ipt
- C:\workspace\Studium\WST\opcua_netzwerk\Entwicklung Knoten\3D Modell\Raspberry Pi 3B\Raspberry Pi 3306.ipt
- C:\workspace\Studium\WST\opcua_netzwerk\Entwicklung Knoten\3D Modell\Raspberry Pi 3B\Raspberry Pi 3307.ipt
- C:\workspace\Studium\WST\opcua_netzwerk\Entwicklung Knoten\3D Modell\Raspberry Pi 3B\Raspberry Pi 3308.ipt
- C:\workspace\Studium\WST\opcua_netzwerk\Entwicklung Knoten\3D Modell\Raspberry Pi 3B\Raspberry Pi 3309.ipt
- C:\workspace\Studium\WST\opcua_netzwerk\Entwicklung Knoten\3D Modell\Raspberry Pi 3B\Raspberry Pi 3310.ipt
- C:\workspace\Studium\WST\opcua_netzwerk\Entwicklung Knoten\3D Modell\Raspberry Pi 3B\Raspberry Pi 3311.ipt
- C:\workspace\Studium\WST\opcua_netzwerk\Entwicklung Knoten\3D Modell\Raspberry Pi 3B\Raspberry Pi 3312.ipt
- C:\workspace\Studium\WST\opcua_netzwerk\Entwicklung Knoten\3D Modell\Raspberry Pi 3B\Raspberry Pi 3313.ipt
- C:\workspace\Studium\WST\opcua_netzwerk\Entwicklung Knoten\3D Modell\Raspberry Pi 3B\Raspberry Pi 3314.ipt
- C:\workspace\Studium\WST\opcua_netzwerk\Entwicklung Knoten\3D Modell\Raspberry Pi 3B\Raspberry Pi 3315.ipt
- C:\workspace\Studium\WST\opcua_netzwerk\Entwicklung Knoten\3D Modell\Raspberry Pi 3B\Raspberry Pi 3316.ipt
- C:\workspace\Studium\WST\opcua_netzwerk\Entwicklung Knoten\3D Modell\Raspberry Pi 3B\Raspberry Pi 3317.ipt
- C:\workspace\Studium\WST\opcua_netzwerk\Entwicklung Knoten\3D Modell\Raspberry Pi 3B\Raspberry Pi 3318.ipt
- C:\workspace\Studium\WST\opcua_netzwerk\Entwicklung Knoten\3D Modell\Raspberry Pi 3B\Raspberry Pi 3319.ipt
- C:\workspace\Studium\WST\opcua_netzwerk\Entwicklung Knoten\3D Modell\Raspberry Pi 3B\Raspberry Pi 3320.ipt
- C:\workspace\Studium\WST\opcua_netzwerk\Entwicklung Knoten\3D Modell\Raspberry Pi 3B\Raspberry Pi 3321.ipt
- C:\workspace\Studium\WST\opcua_netzwerk\Entwicklung Knoten\3D Modell\Raspberry Pi 3B\Raspberry Pi 3322.ipt
- C:\workspace\Studium\WST\opcua_netzwerk\Entwicklung Knoten\3D Modell\Raspberry Pi 3B\Raspberry Pi 3323.ipt
- C:\workspace\Studium\WST\opcua_netzwerk\Entwicklung Knoten\3D Modell\Raspberry Pi 3B\Raspberry Pi 3324.ipt
- C:\workspace\Studium\WST\opcua_netzwerk\Entwicklung Knoten\3D Modell\Raspberry Pi 3B\Raspberry Pi 3325.ipt
- C:\workspace\Studium\WST\opcua_netzwerk\Entwicklung Knoten\3D Modell\Raspberry Pi 3B\Raspberry Pi 3326.ipt
- C:\workspace\Studium\WST\opcua_netzwerk\Entwicklung Knoten\3D Modell\Raspberry Pi 3B\Raspberry Pi 3327.ipt
- C:\workspace\Studium\WST\opcua_netzwerk\Entwicklung Knoten\3D Modell\Raspberry Pi 3B\Raspberry Pi 3328.ipt
- C:\workspace\Studium\WST\opcua_netzwerk\Entwicklung Knoten\3D Modell\Raspberry Pi 3B\Raspberry Pi 3329.ipt
- C:\workspace\Studium\WST\opcua_netzwerk\Entwicklung Knoten\3D Modell\Raspberry Pi 3B\Raspberry Pi 3330.ipt
- C:\workspace\Studium\WST\opcua_netzwerk\Entwicklung Knoten\3D Modell\Raspberry Pi 3B\Raspberry Pi 3331.ipt
- C:\workspace\Studium\WST\opcua_netzwerk\Entwicklung Knoten\3D Modell\Raspberry Pi 3B\Raspberry Pi 3332.ipt
- C:\workspace\Studium\WST\opcua_netzwerk\Entwicklung Knoten\3D Modell\Raspberry Pi 3B\Raspberry Pi 3333.ipt
- C:\workspace\Studium\WST\opcua_netzwerk\Entwicklung Knoten\3D Modell\Raspberry Pi 3B\Raspberry Pi 3334.ipt
- C:\workspace\Studium\WST\opcua_netzwerk\Entwicklung Knoten\3D Modell\Raspberry Pi 3B\Raspberry Pi 3335.ipt
- C:\workspace\Studium\WST\opcua_netzwerk\Entwicklung Knoten\3D Modell\Raspberry Pi 3B\Raspberry Pi 3336.ipt
- C:\workspace\Studium\WST\opcua_netzwerk\Entwicklung Knoten\3D Modell\Raspberry Pi 3B\Raspberry Pi 3337.ipt
- C:\workspace\Studium\WST\opcua_netzwerk\Entwicklung Knoten\3D Modell\Raspberry Pi 3B\Raspberry Pi 3338.ipt
- C:\workspace\Studium\WST\opcua_netzwerk\Entwicklung Knoten\3D Modell\Raspberry Pi 3B\Raspberry Pi 3339.ipt
- C:\workspace\Studium\WST\opcua_netzwerk\Entwicklung Knoten\3D Modell\Raspberry Pi 3B\Raspberry Pi 3340.ipt
- C:\workspace\Studium\WST\opcua_netzwerk\Entwicklung Knoten\3D Modell\Raspberry Pi 3B\Raspberry Pi 3341.ipt
- C:\workspace\Studium\WST\opcua_netzwerk\Entwicklung Knoten\3D Modell\Raspberry Pi 3B\Raspberry Pi 3342.ipt
- C:\workspace\Studium\WST\opcua_netzwerk\Entwicklung Knoten\3D Modell\Raspberry Pi 3B\Raspberry Pi 3343.ipt
- C:\workspace\Studium\WST\opcua_netzwerk\Entwicklung Knoten\3D Modell\Raspberry Pi 3B\Raspberry Pi 3344.ipt
- C:\workspace\Studium\WST\opcua_netzwerk\Entwicklung Knoten\3D Modell\Raspberry Pi 3B\Raspberry Pi 3345.ipt
- C:\workspace\Studium\WST\opcua_netzwerk\Entwicklung Knoten\3D Modell\Raspberry Pi 3B\Raspberry Pi 3346.ipt
- C:\workspace\Studium\WST\opcua_netzwerk\Entwicklung Knoten\3D Modell\Raspberry Pi 3B\Raspberry Pi 3347.ipt
- C:\workspace\Studium\WST\opcua_netzwerk\Entwicklung Knoten\3D Modell\Raspberry Pi 3B\Raspberry Pi 3348.ipt
- C:\workspace\Studium\WST\opcua_netzwerk\Entwicklung Knoten\3D Modell\Raspberry Pi 3B\Raspberry Pi 3349.ipt
- C:\workspace\Studium\WST\opcua_netzwerk\Entwicklung Knoten\3D Modell\Raspberry Pi 3B\Raspberry Pi 3350.ipt
- C:\workspace\Studium\WST\opcua_netzwerk\Entwicklung Knoten\3D Modell\Raspberry Pi 3B\Raspberry Pi 3351.ipt
- C:\workspace\Studium\WST\opcua_netzwerk\Entwicklung Knoten\3D Modell\Raspberry Pi 3B\Raspberry Pi 3352.ipt
- C:\workspace\Studium\WST\opcua_netzwerk\Entwicklung Knoten\3D Modell\Raspberry Pi 3B\Raspberry Pi 3353.ipt
- C:\workspace\Studium\WST\opcua_netzwerk\Entwicklung Knoten\3D Modell\Raspberry Pi 3B\Raspberry Pi 3354.ipt
- C:\workspace\Studium\WST\opcua_netzwerk\Entwicklung Knoten\3D Modell\Raspberry Pi 3B\Raspberry Pi 3357.ipt
- C:\workspace\Studium\WST\opcua_netzwerk\Entwicklung Knoten\3D Modell\Raspberry Pi 3B\Raspberry Pi 3355.ipt
- C:\workspace\Studium\WST\opcua_netzwerk\Entwicklung Knoten\3D Modell\Raspberry Pi 3B\Raspberry Pi 3356.ipt
- C:\workspace\Studium\WST\opcua_netzwerk\Entwicklung Knoten\3D Modell\Raspberry Pi 3B\Part2^Raspberry Pi 3.ipt
- C:\workspace\Studium\WST\opcua_netzwerk\Entwicklung Knoten\3D Modell\Raspberry Pi 3B\Raspberry Pi 3360.ipt
- C:\workspace\Studium\WST\opcua_netzwerk\Entwicklung Knoten\3D Modell\Raspberry Pi 3B\Part4^Raspberry Pi 3.ipt
- C:\workspace\Studium\WST\opcua_netzwerk\Entwicklung Knoten\3D Modell\Raspberry Pi 3B\Solder2.ipt
- C:\workspace\Studium\WST\opcua_netzwerk\Entwicklung Knoten\3D Modell\Raspberry Pi 3B\Raspberry Pi 3359.ipt
- C:\workspace\Studium\WST\opcua_netzwerk\Entwicklung Knoten\3D Modell\Raspberry Pi 3B\mf-msmf050-2.ipt
- C:\workspace\Studium\WST\opcua_netzwerk\Entwicklung Knoten\3D Modell\Raspberry Pi 3B\Raspberry Pi 3163_smaller.ipt
- C:\workspace\Studium\WST\opcua_netzwerk\Entwicklung Knoten\3D Modell\Raspberry Pi 3B\Raspberry Pi 353_smaller.ipt
- C:\workspace\Studium\WST\opcua_netzwerk\Entwicklung Knoten\3D Modell\Raspberry Pi 3B\Raspberry Pi 3164_small.ipt
- C:\workspace\Studium\WST\opcua_netzwerk\Entwicklung Knoten\3D Modell\Raspberry Pi 3B\Raspberry Pi 3165_smaller.ipt
- C:\workspace\Studium\WST\opcua_netzwerk\Entwicklung Knoten\3D Modell\Raspberry Pi 3B\Raspberry Pi 3141_smaller.ipt
- C:\workspace\Studium\WST\opcua_netzwerk\Entwicklung Knoten\3D Modell\Raspberry Pi 3B\raspberry_pi_B+_(microsd2).ipt
- C:\workspace\Studium\WST\opcua_netzwerk\Entwicklung Knoten\3D Modell\Raspberry Pi 3B\raspberry_pi_B_(RJ45).ipt
## Components (633 placed, 633 different names)
1. Raspberry Pi 3157_1
2. Raspberry Pi 3242_2
3. Raspberry Pi 3266_3
4. raspberry_pi_3(bar_180_2x20)_4
5. RPi3_ModelB v1_5 [sub-assembly]
6. Raspberry Pi 312_6
7. Raspberry Pi 314_7
8. Raspberry Pi 3172_8
9. Raspberry Pi 3173_9
10. Raspberry Pi 3174_10
11. Raspberry Pi 3175_11
12. Raspberry Pi 3176_12
13. Raspberry Pi 3177_13
14. Raspberry Pi 3178_14
15. Raspberry Pi 3179_15
16. Raspberry Pi 3180_16
17. Raspberry Pi 3181_17
18. Raspberry Pi 3182_18
19. Raspberry Pi 3183_19
20. Raspberry Pi 3184_20
21. Raspberry Pi 3185_21
22. Raspberry Pi 3186_22
23. Raspberry Pi 3187_23
24. Raspberry Pi 3188_24
25. Raspberry Pi 3189_25
26. Raspberry Pi 3190_26
27. Raspberry Pi 3191_27
28. Raspberry Pi 3192_28
29. Raspberry Pi 3193_29
30. Raspberry Pi 3194_30
31. Raspberry Pi 3195_31
32. Raspberry Pi 3196_32
33. Raspberry Pi 3197_33
34. Raspberry Pi 3198_34
35. Raspberry Pi 3199_35
36. Raspberry Pi 3200_36
37. Raspberry Pi 3201_37
38. Raspberry Pi 3202_38
39. Raspberry Pi 3203_39
40. Raspberry Pi 3204_40
41. Raspberry Pi 3205_41
42. Raspberry Pi 3206_42
43. Raspberry Pi 3207_43
44. Raspberry Pi 3208_44
45. Raspberry Pi 3209_45
46. Raspberry Pi 3210_46
47. Raspberry Pi 3211_47
48. Raspberry Pi 3212_48
49. Raspberry Pi 3213_49
50. Raspberry Pi 3214_50
51. Raspberry Pi 3215_51
52. Raspberry Pi 3216_52
53. Raspberry Pi 3217_53
54. Raspberry Pi 3218_54
55. Raspberry Pi 3219_55
56. Raspberry Pi 3220_56
57. Raspberry Pi 3221_57
58. Raspberry Pi 3222_58
59. Raspberry Pi 3223_59
60. Raspberry Pi 3224_60
61. Raspberry Pi 3225_61
62. Raspberry Pi 3226_62
63. Raspberry Pi 3227_63
64. Raspberry Pi 3228_64
65. Raspberry Pi 3229_65
66. Raspberry Pi 3230_66
67. Raspberry Pi 3231_67
68. Raspberry Pi 3232_68
69. Raspberry Pi 3233_69
70. Raspberry Pi 3234_70
71. Raspberry Pi 3235_71
72. Raspberry Pi 31_72
73. Raspberry Pi 32_73
74. Raspberry Pi 33_74
75. Raspberry Pi 34_75
76. Raspberry Pi 35_76
77. Raspberry Pi 36_77
78. Raspberry Pi 37_78
79. Raspberry Pi 38_79
80. Raspberry Pi 39_80
81. Raspberry Pi 310_81
82. Raspberry Pi 311_82
83. Raspberry Pi 313_83
84. Raspberry Pi 315_84
85. Raspberry Pi 316_85
86. Raspberry Pi 317_86
87. Raspberry Pi 318_87
88. Raspberry Pi 319_88
89. Raspberry Pi 320_89
90. Raspberry Pi 322_90
91. Raspberry Pi 323_91
92. Raspberry Pi 324_92
93. Raspberry Pi 325_93
94. Raspberry Pi 326_94
95. Raspberry Pi 327_95
96. Raspberry Pi 328_96
97. Raspberry Pi 329_97
98. Raspberry Pi 330_98
99. Raspberry Pi 331_99
100. Raspberry Pi 332_100
101. Raspberry Pi 333_101
102. Raspberry Pi 334_102
103. Raspberry Pi 335_103
104. Raspberry Pi 336_104
105. Raspberry Pi 337_105
106. Raspberry Pi 338_106
107. Raspberry Pi 339_107
108. Raspberry Pi 340_108
109. Raspberry Pi 341_109
110. Raspberry Pi 342_110
111. Raspberry Pi 343_111
112. Raspberry Pi 344_112
113. Raspberry Pi 345_113
114. Raspberry Pi 346_114
115. Raspberry Pi 347_115
116. Raspberry Pi 348_116
117. Raspberry Pi 349_117
118. Raspberry Pi 350_118
119. Raspberry Pi 351_119
120. Raspberry Pi 352_120
121. Raspberry Pi 353_121
122. Raspberry Pi 354_122
123. Raspberry Pi 355_123
124. Raspberry Pi 356_124
125. Raspberry Pi 357_125
126. Raspberry Pi 358_126
127. Raspberry Pi 359_127
128. Raspberry Pi 360_128
129. Raspberry Pi 361_129
130. Raspberry Pi 362_130
131. Raspberry Pi 363_131
132. Raspberry Pi 364_132
133. Raspberry Pi 365_133
134. Raspberry Pi 366_134
135. Raspberry Pi 367_135
136. Raspberry Pi 368_136
137. Raspberry Pi 369_137
138. Raspberry Pi 370_138
139. Raspberry Pi 371_139
140. Raspberry Pi 372_140
141. Raspberry Pi 373_141
142. Raspberry Pi 374_142
143. Raspberry Pi 375_143
144. Raspberry Pi 376_144
145. Raspberry Pi 377_145
146. Raspberry Pi 378_146
147. Raspberry Pi 379_147
148. Raspberry Pi 380_148
149. Raspberry Pi 381_149
150. Raspberry Pi 382_150
151. Raspberry Pi 383_151
152. Raspberry Pi 385_152
153. Raspberry Pi 386_153
154. Raspberry Pi 387_154
155. Raspberry Pi 388_155
156. Raspberry Pi 390_156
157. Raspberry Pi 391_157
158. Raspberry Pi 393_158
159. Raspberry Pi 394_159
160. Raspberry Pi 395_160
161. Raspberry Pi 396_161
162. Raspberry Pi 397_162
163. Raspberry Pi 398_163
164. Raspberry Pi 399_164
165. Raspberry Pi 3100_165
166. Raspberry Pi 3101_166
167. Raspberry Pi 3102_167
168. Raspberry Pi 3103_168
169. Raspberry Pi 3104_169
170. Raspberry Pi 3105_170
171. Raspberry Pi 3106_171
172. Raspberry Pi 3107_172
173. Raspberry Pi 3108_173
174. Raspberry Pi 3109_174
175. Raspberry Pi 3110_175
176. Raspberry Pi 3111_176
177. Raspberry Pi 3112_177
178. Raspberry Pi 3113_178
179. Raspberry Pi 3114_179
180. Raspberry Pi 3115_180
181. Raspberry Pi 3116_181
182. Raspberry Pi 3117_182
183. Raspberry Pi 3118_183
184. Raspberry Pi 3119_184
185. Raspberry Pi 3120_185
186. Raspberry Pi 3121_186
187. Raspberry Pi 3122_187
188. Raspberry Pi 3123_188
189. Raspberry Pi 3124_189
190. Raspberry Pi 3125_190
191. Raspberry Pi 3126_191
192. Raspberry Pi 3127_192
193. Raspberry Pi 3128_193
194. Raspberry Pi 3129_194
195. Raspberry Pi 3130_195
196. Raspberry Pi 3131_196
197. Raspberry Pi 3132_197
198. Raspberry Pi 3133_198
199. Raspberry Pi 3134_199
200. Raspberry Pi 3135_200
201. Raspberry Pi 3137_201
202. Raspberry Pi 3138_202
203. Raspberry Pi 3139_203
204. Raspberry Pi 3140_204
205. Raspberry Pi 3141_205
206. Raspberry Pi 3142_206
207. Raspberry Pi 3143_207
208. Raspberry Pi 3144_208
209. Raspberry Pi 3146_209
210. Raspberry Pi 3147_210
211. Raspberry Pi 3149_211
212. Raspberry Pi 3150_212
213. Raspberry Pi 3151_213
214. Raspberry Pi 3152_214
215. Raspberry Pi 3153_215
216. Raspberry Pi 3154_216
217. Raspberry Pi 3155_217
218. Raspberry Pi 3156_218
219. Raspberry Pi 3158_219
220. Raspberry Pi 3159_220
221. Raspberry Pi 3160_221
222. Raspberry Pi 3161_222
223. Raspberry Pi 3162_223
224. Raspberry Pi 3163_224
225. Raspberry Pi 3164_225
226. Raspberry Pi 3165_226
227. Raspberry Pi 3166_227
228. Raspberry Pi 3167_228
229. Raspberry Pi 3168_229
230. Raspberry Pi 3169_230
231. Raspberry Pi 3170_231
232. Raspberry Pi 3171_232
233. Raspberry Pi 3276_233
234. Raspberry Pi 3277_234
235. Raspberry Pi 3278_235
236. Raspberry Pi 3279_236
237. Raspberry Pi 3280_237
238. Raspberry Pi 3281_238
239. Raspberry Pi 3282_239
240. Raspberry Pi 3283_240
241. Raspberry Pi 3284_241
242. Raspberry Pi 3285_242
243. Raspberry Pi 3286_243
244. Raspberry Pi 3287_244
245. Raspberry Pi 3288_245
246. Raspberry Pi 3289_246
247. Raspberry Pi 3290_247
248. Raspberry Pi 3291_248
249. Raspberry Pi 3292_249
250. Raspberry Pi 3293_250
251. Raspberry Pi 3294_251
252. Raspberry Pi 3295_252
253. Raspberry Pi 3296_253
254. Raspberry Pi 3297_254
255. Raspberry Pi 3298_255
256. Raspberry Pi 3299_256
257. Raspberry Pi 3300_257
258. Raspberry Pi 3301_258
259. Raspberry Pi 3302_259
260. Raspberry Pi 3303_260
261. Raspberry Pi 3304_261
262. Raspberry Pi 3305_262
263. Raspberry Pi 3306_263
264. Raspberry Pi 3307_264
265. Raspberry Pi 3308_265
266. Raspberry Pi 3309_266
267. Raspberry Pi 3310_267
268. Raspberry Pi 3311_268
269. Raspberry Pi 3312_269
270. Raspberry Pi 3313_270
271. Raspberry Pi 3314_271
272. Raspberry Pi 3315_272
273. Raspberry Pi 3316_273
274. Raspberry Pi 3317_274
275. Raspberry Pi 3318_275
276. Raspberry Pi 3319_276
277. Raspberry Pi 3320_277
278. Raspberry Pi 3321_278
279. Raspberry Pi 3322_279
280. Raspberry Pi 3323_280
281. Raspberry Pi 3324_281
282. Raspberry Pi 3325_282
283. Raspberry Pi 3326_283
284. Raspberry Pi 3327_284
285. Raspberry Pi 3328_285
286. Raspberry Pi 3329_286
287. Raspberry Pi 3330_287
288. Raspberry Pi 3331_288
289. Raspberry Pi 3332_289
290. Raspberry Pi 3333_290
291. Raspberry Pi 3334_291
292. Raspberry Pi 3335_292
293. Raspberry Pi 3336_293
294. Raspberry Pi 3337_294
295. Raspberry Pi 3338_295
296. Raspberry Pi 3339_296
297. Raspberry Pi 3340_297
298. Raspberry Pi 3341_298
299. Raspberry Pi 3342_299
300. Raspberry Pi 3343_300
301. Raspberry Pi 3344_301
302. Raspberry Pi 3345_302
303. Raspberry Pi 3346_303
304. Raspberry Pi 3347_304
305. Raspberry Pi 3348_305
306. Raspberry Pi 3349_306
307. Raspberry Pi 3350_307
308. Raspberry Pi 3351_308
309. Raspberry Pi 3352_309
310. Raspberry Pi 3353_310
311. Raspberry Pi 3354_311
312. Raspberry Pi 327_312
313. Raspberry Pi 340_313
314. Raspberry Pi 344_314
315. Raspberry Pi 344_315
316. Raspberry Pi 340_316
317. Raspberry Pi 344_317
318. Raspberry Pi 340_318
319. Raspberry Pi 344_319
320. Raspberry Pi 340_320
321. Raspberry Pi 344_321
322. Raspberry Pi 340_322
323. Raspberry Pi 340_323
324. Raspberry Pi 344_324
325. Raspberry Pi 340_325
326. Raspberry Pi 344_326
327. Raspberry Pi 3357_327
328. Raspberry Pi 3355_328
329. Raspberry Pi 3356_329
330. Raspberry Pi 374_330
331. Raspberry Pi 3141_331
332. Raspberry Pi 374_332
333. Raspberry Pi 374_333
334. Raspberry Pi 374_334
335. Part2^Raspberry Pi 3_335
336. Raspberry Pi 3360_336
337. Part4^Raspberry Pi 3_337
338. Raspberry Pi 3159_338
339. Raspberry Pi 3158_339
340. Raspberry Pi 3160_340
341. Raspberry Pi 3162_341
342. Raspberry Pi 3161_342
343. Raspberry Pi 359_343
344. Raspberry Pi 3165_344
345. Raspberry Pi 353_345
346. Raspberry Pi 3164_346
347. Raspberry Pi 3163_347
348. Raspberry Pi 355_348
349. Raspberry Pi 3168_349
350. Raspberry Pi 3170_350
351. Raspberry Pi 3169_351
352. Raspberry Pi 3171_352
353. Raspberry Pi 3167_353
354. Raspberry Pi 3166_354
355. Raspberry Pi 353_355
356. Raspberry Pi 3165_356
357. Raspberry Pi 3163_357
358. Raspberry Pi 3164_358
359. Solder2_359
360. Solder2_360
361. Solder2_361
362. Solder2_362
363. Solder2_363
364. Solder2_364
365. Solder2_365
366. Solder2_366
367. Solder2_367
368. Solder2_368
369. Solder2_369
370. Raspberry Pi 3359_370
371. Solder2_371
372. Solder2_372
373. Solder2_373
374. Solder2_374
375. Solder2_375
376. Solder2_376
377. Solder2_377
378. Solder2_378
379. Solder2_379
380. Solder2_380
381. Solder2_381
382. Solder2_382
383. mf-msmf050-2_383
384. Solder2_384
385. Raspberry Pi 3163_smaller_385
386. Raspberry Pi 353_smaller_386
387. Raspberry Pi 3164_small_387
388. Raspberry Pi 3165_smaller_388
389. Raspberry Pi 3163_smaller_389
390. Raspberry Pi 353_smaller_390
391. Raspberry Pi 3164_small_391
392. Raspberry Pi 3165_smaller_392
393. Raspberry Pi 3163_smaller_393
394. Raspberry Pi 353_smaller_394
395. Raspberry Pi 3164_small_395
396. Raspberry Pi 3165_smaller_396
397. Raspberry Pi 3141_397
398. Raspberry Pi 3141_398
399. Raspberry Pi 3141_399
400. Raspberry Pi 3141_400
401. Raspberry Pi 3141_401
402. Raspberry Pi 3141_402
403. Raspberry Pi 3141_403
404. Raspberry Pi 3141_404
405. Raspberry Pi 3141_405
406. Raspberry Pi 3141_406
407. Raspberry Pi 3141_407
408. Raspberry Pi 3141_408
409. Raspberry Pi 3141_409
410. Raspberry Pi 3141_410
411. Raspberry Pi 3141_411
412. Raspberry Pi 3141_412
413. Raspberry Pi 3141_413
414. Raspberry Pi 3141_414
415. Raspberry Pi 3141_415
416. Raspberry Pi 3141_416
417. Raspberry Pi 3141_417
418. Raspberry Pi 3141_418
419. Raspberry Pi 3141_419
420. Raspberry Pi 3141_420
421. Raspberry Pi 3141_421
422. Raspberry Pi 3141_422
423. Raspberry Pi 3141_423
424. Raspberry Pi 3141_424
425. Raspberry Pi 3141_425
426. Raspberry Pi 3141_426
427. Raspberry Pi 3141_427
428. Raspberry Pi 3141_428
429. Raspberry Pi 3141_429
430. Raspberry Pi 3141_430
431. Raspberry Pi 3141_431
432. Raspberry Pi 3141_432
433. Raspberry Pi 3141_433
434. Raspberry Pi 3141_434
435. Raspberry Pi 3141_435
436. Raspberry Pi 3141_436
437. Raspberry Pi 3141_437
438. Raspberry Pi 3141_438
439. Raspberry Pi 3141_439
440. Raspberry Pi 3141_440
441. Raspberry Pi 3141_441
442. Raspberry Pi 3141_442
443. Raspberry Pi 3141_443
444. Raspberry Pi 3141_444
445. Raspberry Pi 3141_445
446. Raspberry Pi 3141_446
447. Raspberry Pi 3141_447
448. Raspberry Pi 3141_448
449. Raspberry Pi 3141_449
450. Raspberry Pi 3141_450
451. Raspberry Pi 3141_451
452. Raspberry Pi 3141_452
453. Raspberry Pi 3141_453
454. Raspberry Pi 3141_454
455. Raspberry Pi 374_455
456. Raspberry Pi 3141_456
457. Raspberry Pi 3141_457
458. Raspberry Pi 3141_458
459. Raspberry Pi 3141_459
460. Raspberry Pi 3141_460
461. Raspberry Pi 3141_461
462. Raspberry Pi 3141_462
463. Raspberry Pi 3141_463
464. Raspberry Pi 3141_464
465. Raspberry Pi 3141_465
466. Raspberry Pi 3141_466
467. Raspberry Pi 3141_467
468. Raspberry Pi 3141_468
469. Raspberry Pi 3141_469
470. Raspberry Pi 3141_470
471. Raspberry Pi 3141_471
472. Raspberry Pi 3141_472
473. Raspberry Pi 3141_473
474. Raspberry Pi 3141_474
475. Raspberry Pi 3141_475
476. Raspberry Pi 3141_476
477. Raspberry Pi 3141_477
478. Raspberry Pi 3141_478
479. Raspberry Pi 3141_479
480. Raspberry Pi 3141_480
481. Raspberry Pi 3141_481
482. Raspberry Pi 3141_482
483. Raspberry Pi 3141_smaller_483
484. Raspberry Pi 3141_smaller_484
485. Raspberry Pi 3141_smaller_485
486. Raspberry Pi 3141_smaller_486
487. Raspberry Pi 3141_smaller_487
488. Raspberry Pi 3141_smaller_488
489. Raspberry Pi 3141_smaller_489
490. Raspberry Pi 3141_smaller_490
491. Raspberry Pi 3141_smaller_491
492. Raspberry Pi 3141_smaller_492
493. Raspberry Pi 3141_smaller_493
494. Raspberry Pi 3141_smaller_494
495. Raspberry Pi 3141_smaller_495
496. Raspberry Pi 3141_smaller_496
497. Raspberry Pi 3141_smaller_497
498. Raspberry Pi 3141_smaller_498
499. Raspberry Pi 3141_smaller_499
500. Raspberry Pi 3141_smaller_500
501. Raspberry Pi 3141_smaller_501
502. Raspberry Pi 3141_smaller_502
503. Raspberry Pi 3141_smaller_503
504. Raspberry Pi 3141_smaller_504
505. Raspberry Pi 3141_smaller_505
506. Raspberry Pi 3141_smaller_506
507. Raspberry Pi 3141_smaller_507
508. Raspberry Pi 3281_508
509. Raspberry Pi 3280_509
510. Raspberry Pi 3282_510
511. Raspberry Pi 3285_511
512. Raspberry Pi 3283_512
513. Raspberry Pi 3284_513
514. Raspberry Pi 34_514
515. Raspberry Pi 3141_smaller_515
516. Raspberry Pi 3141_smaller_516